# Autodesk Inventor assembly: double_spool_6mm_clamping_hubAssembly
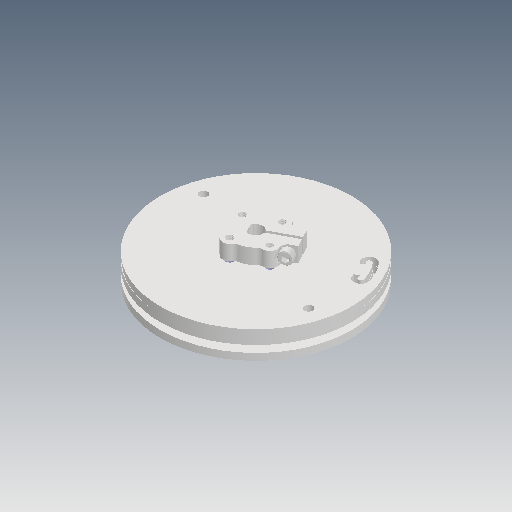
[picture p0: Inventor's stored thumbnail of the model, 512x512]
Saved by Autodesk Inventor 2020 (Build 240168000, 168)
## iProperties
Created: 2019-11-26
Part Number: double_spool_6mm_clamping_hubAssembly
Document SubType Name: Assembly
Designer: ball
Author: ball
## Documents named in this file (3)
- C:\FTC\FTC8863CAD\2019 Robot\Delivery\double_spool_6mm_clamping_hubAssembly.iam
- C:\FTC\FTC8863CAD\Actobotics\615 parts\615468_double_spool_Assembly.iam
- C:\FTC\FTC8863CAD\Actobotics\545 parts\545619 assembly.ipt
## Components (2 placed, 2 different names)
1. 615468_double_spool_Assembly:1 [sub-assembly] — Mate:1, Mate:2, Mate:3, Mate:4
2. 545619 assembly:1 — Mate:1, Mate:2, Mate:3, Mate:4
## Relationships (4: Mate 4)
- Mate:1: 615468_double_spool_Assembly:1 ↔ 545619 assembly:1
- Mate:2: 615468_double_spool_Assembly:1 ↔ 545619 assembly:1
- Mate:3: 615468_double_spool_Assembly:1 ↔ 545619 assembly:1
- Mate:4: 615468_double_spool_Assembly:1 ↔ 545619 assembly:1
